# Autodesk Inventor assembly: ASY MSC 800 gills
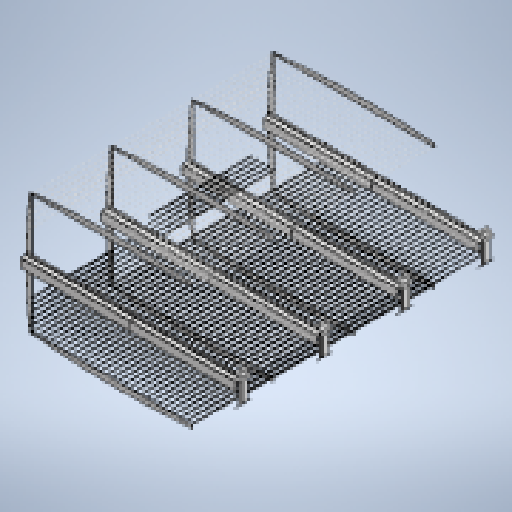
[picture p0: Inventor's stored thumbnail of the model, 512x512]
Saved by Autodesk Inventor 2025 (Build 290162010, 162A)
## iProperties
Created: 2024-08-31
Part Number: ASY MSC 800 gills
Document SubType Name: Assembly
Designer: pokla
Stock Number: ASY МОО 800 Жабры
Mass: 469810 g
Surface Area: 1.86943e+06 cm^2
Volume: 67870.7 cm^3
Density: 6.92212 g/cm^3
Author: pokla
## Documents named in this file (14)
- C:\Users\admin\YandexDisk-badmisterfox\домашниий пк\Inventor\Manturovo\Manturovo_Se-clar\ASY MSC 800 gills.iam
- C:\Users\admin\YandexDisk-badmisterfox\домашниий пк\Inventor\Manturovo\Manturovo_Se-clar\MSC 804 sheet gills.ipt
- C:\Users\admin\YandexDisk-badmisterfox\домашниий пк\Inventor\Manturovo\Manturovo_Se-clar\MSC 810 pillar gills.ipt
- C:\Users\admin\YandexDisk-badmisterfox\домашниий пк\Inventor\Manturovo\Manturovo_Se-clar\MSC 805 sheet gills.ipt
- C:\Users\admin\YandexDisk-badmisterfox\домашниий пк\Inventor\Manturovo\Manturovo_Se-clar\MSC 806 sheet gills.ipt
- C:\Users\admin\YandexDisk-badmisterfox\домашниий пк\Inventor\Manturovo\Manturovo_Se-clar\MSC 807 sheet gills.ipt
- C:\Users\admin\YandexDisk-badmisterfox\домашниий пк\Inventor\Manturovo\Manturovo_Se-clar\MSC 808 sheet gills.ipt
- C:\Users\admin\YandexDisk-badmisterfox\домашниий пк\Inventor\Manturovo\Manturovo_Se-clar\MSC 809 sheet gills.ipt
- C:\Users\admin\YandexDisk-badmisterfox\домашниий пк\Inventor\Manturovo\Manturovo_Se-clar\MSC 813 wall support gills.ipt
- C:\Users\admin\YandexDisk-badmisterfox\домашниий пк\Inventor\Manturovo\Manturovo_Se-clar\MSC 811 pillar gills.ipt
- C:\Users\admin\YandexDisk-badmisterfox\домашниий пк\Inventor\Manturovo\Manturovo_Se-clar\MSC 814 string for sheets gills.ipt
- C:\Users\admin\YandexDisk-badmisterfox\домашниий пк\Inventor\Manturovo\Manturovo_Se-clar\MSC 812 top support gills.ipt
- C:\Users\admin\YandexDisk-badmisterfox\домашниий пк\Inventor\Manturovo\Manturovo_Se-clar\MSC 803 sheet gills.ipt
- C:\Users\admin\YandexDisk-badmisterfox\домашниий пк\Inventor\Manturovo\Manturovo_Se-clar\ASY MSC 800.1 gills base.iam
## Components (272 placed, 13 different names)
1. MSC 0203 sheet gills:1 — Angle:2, Tangent:8, Tangent:9, Flush:15, Flush:19
2. MSC 0204 sheet gills:1 — Angle:3, Tangent:10, Tangent:11, Flush:15, Flush:16
3. MSC 0205 sheet gills:1 — Angle:4, Tangent:12, Tangent:13, Flush:16, Flush:17
4. MSC 0206 sheet gills:1 — Angle:5, Tangent:17, Tangent:18, Flush:17, Flush:18
5. MSC 0207 sheet gills:1 — Angle:6, Tangent:19, Tangent:20, Flush:18
6. MSC 814 string for sheets gills:143 — Rigid:40
7. MSC 814 string for sheets gills:152 — Rigid:24
8. MSC 814 string for sheets gills:371
9. MSC 814 string for sheets gills:372
10. MSC 814 string for sheets gills:373
11. MSC 814 string for sheets gills:374
12. MSC 814 string for sheets gills:375
13. MSC 814 string for sheets gills:2 — Rigid:12
14. MSC 0201 sheet gills:1 — Rigid:33, Angle:2, Angle:3, Angle:4, Angle:5, Angle:6, Tangent:14, Tangent:15, Tangent:16, Flush:19, Flush:24
15. MSC 804 sheet gills:1 — Rigid:33
16. MSC 814 string for sheets gills:1 — Rotational:1
17. MSC 814 string for sheets gills:3 — Rotational:2, Tangent:23
18. MSC 814 string for sheets gills:376 — Rotational:3, Tangent:21, Tangent:22
19. MSC 0201 sheet gills:30 — Tangent:21, Tangent:23, Flush:24
20. MSC 804 sheet gills:30 — Tangent:22
21. MSC 814 string for sheets gills:377
22. MSC 0201 sheet gills:2
23. MSC 804 sheet gills:2
24. MSC 814 string for sheets gills:378
25. MSC 814 string for sheets gills:379
26. MSC 814 string for sheets gills:380
27. MSC 0201 sheet gills:31
28. MSC 804 sheet gills:31
29. MSC 814 string for sheets gills:381
30. MSC 0201 sheet gills:3
31. MSC 804 sheet gills:3
32. MSC 814 string for sheets gills:382
33. MSC 814 string for sheets gills:383
34. MSC 814 string for sheets gills:384
35. MSC 0201 sheet gills:32
36. MSC 804 sheet gills:32
37. MSC 814 string for sheets gills:385
38. MSC 0201 sheet gills:4
39. MSC 804 sheet gills:4
40. MSC 814 string for sheets gills:386
41. MSC 814 string for sheets gills:387
42. MSC 814 string for sheets gills:388
43. MSC 0201 sheet gills:33
44. MSC 804 sheet gills:33
45. MSC 814 string for sheets gills:389
46. MSC 0201 sheet gills:5
47. MSC 804 sheet gills:5
48. MSC 814 string for sheets gills:390
49. MSC 814 string for sheets gills:391
50. MSC 814 string for sheets gills:392
51. MSC 0201 sheet gills:34
52. MSC 804 sheet gills:34
53. MSC 814 string for sheets gills:393
54. MSC 0201 sheet gills:6
55. MSC 804 sheet gills:6
56. MSC 814 string for sheets gills:394
57. MSC 814 string for sheets gills:395
58. MSC 814 string for sheets gills:396
59. MSC 0201 sheet gills:35
60. MSC 804 sheet gills:35
61. MSC 814 string for sheets gills:397
62. MSC 0201 sheet gills:7
63. MSC 804 sheet gills:7
64. MSC 814 string for sheets gills:398
65. MSC 814 string for sheets gills:399
66. MSC 814 string for sheets gills:400
67. MSC 0201 sheet gills:36
68. MSC 804 sheet gills:36
69. MSC 814 string for sheets gills:401
70. MSC 0201 sheet gills:8
71. MSC 804 sheet gills:8
72. MSC 814 string for sheets gills:402
73. MSC 814 string for sheets gills:403
74. MSC 814 string for sheets gills:404
75. MSC 0201 sheet gills:37
76. MSC 804 sheet gills:37
77. MSC 814 string for sheets gills:405
78. MSC 0201 sheet gills:9
79. MSC 804 sheet gills:9
80. MSC 814 string for sheets gills:406
81. MSC 814 string for sheets gills:407
82. MSC 814 string for sheets gills:408
83. MSC 0201 sheet gills:38
84. MSC 804 sheet gills:38
85. MSC 814 string for sheets gills:409
86. MSC 0201 sheet gills:10
87. MSC 804 sheet gills:10
88. MSC 814 string for sheets gills:410
89. MSC 814 string for sheets gills:411
90. MSC 814 string for sheets gills:412
91. MSC 0201 sheet gills:39
92. MSC 804 sheet gills:39
93. MSC 814 string for sheets gills:413
94. MSC 0201 sheet gills:11
95. MSC 804 sheet gills:11
96. MSC 814 string for sheets gills:414
97. MSC 814 string for sheets gills:415
98. MSC 814 string for sheets gills:416
99. MSC 0201 sheet gills:40
100. MSC 804 sheet gills:40
101. MSC 814 string for sheets gills:417
102. MSC 0201 sheet gills:12
103. MSC 804 sheet gills:12
104. MSC 814 string for sheets gills:418
105. MSC 814 string for sheets gills:419
106. MSC 814 string for sheets gills:420
107. MSC 0201 sheet gills:41
108. MSC 804 sheet gills:41
109. MSC 814 string for sheets gills:421
110. MSC 0201 sheet gills:13
111. MSC 804 sheet gills:13
112. MSC 814 string for sheets gills:422
113. MSC 814 string for sheets gills:423
114. MSC 814 string for sheets gills:424
115. MSC 0201 sheet gills:42
116. MSC 804 sheet gills:42
117. MSC 814 string for sheets gills:425
118. MSC 0201 sheet gills:14
119. MSC 804 sheet gills:14
120. MSC 814 string for sheets gills:426
121. MSC 814 string for sheets gills:427
122. MSC 814 string for sheets gills:428
123. MSC 0201 sheet gills:43
124. MSC 804 sheet gills:43
125. MSC 814 string for sheets gills:429
126. MSC 0201 sheet gills:15
127. MSC 804 sheet gills:15
128. MSC 814 string for sheets gills:430
129. MSC 814 string for sheets gills:431
130. MSC 814 string for sheets gills:432
131. MSC 0201 sheet gills:44
132. MSC 804 sheet gills:44
133. MSC 814 string for sheets gills:433
134. MSC 0201 sheet gills:16
135. MSC 804 sheet gills:16
136. MSC 814 string for sheets gills:434
137. MSC 814 string for sheets gills:435
138. MSC 814 string for sheets gills:436
139. MSC 0201 sheet gills:45
140. MSC 804 sheet gills:45
141. MSC 814 string for sheets gills:437
142. MSC 0201 sheet gills:17
143. MSC 804 sheet gills:17
144. MSC 814 string for sheets gills:438
145. MSC 814 string for sheets gills:439
146. MSC 814 string for sheets gills:440
147. MSC 0201 sheet gills:46
148. MSC 804 sheet gills:46
149. MSC 814 string for sheets gills:441
150. MSC 0201 sheet gills:18
151. MSC 804 sheet gills:18
152. MSC 814 string for sheets gills:442
153. MSC 814 string for sheets gills:443
154. MSC 814 string for sheets gills:444
155. MSC 0201 sheet gills:47
156. MSC 804 sheet gills:47
157. MSC 814 string for sheets gills:445
158. MSC 0201 sheet gills:19
159. MSC 804 sheet gills:19
160. MSC 814 string for sheets gills:446
161. MSC 814 string for sheets gills:447
162. MSC 814 string for sheets gills:448
163. MSC 0201 sheet gills:48
164. MSC 804 sheet gills:48
165. MSC 814 string for sheets gills:449
166. MSC 0201 sheet gills:20
167. MSC 804 sheet gills:20
168. MSC 814 string for sheets gills:450
169. MSC 814 string for sheets gills:451
170. MSC 814 string for sheets gills:452
171. MSC 0201 sheet gills:49
172. MSC 804 sheet gills:49
173. MSC 814 string for sheets gills:453
174. MSC 0201 sheet gills:21
175. MSC 804 sheet gills:21
176. MSC 814 string for sheets gills:454
177. MSC 814 string for sheets gills:455
178. MSC 814 string for sheets gills:456
179. MSC 0201 sheet gills:50
180. MSC 804 sheet gills:50
181. MSC 814 string for sheets gills:457
182. MSC 0201 sheet gills:22
183. MSC 804 sheet gills:22
184. MSC 814 string for sheets gills:458
185. MSC 814 string for sheets gills:459
186. MSC 814 string for sheets gills:460
187. MSC 0201 sheet gills:51
188. MSC 804 sheet gills:51
189. MSC 814 string for sheets gills:461
190. MSC 0201 sheet gills:23
191. MSC 804 sheet gills:23
192. MSC 814 string for sheets gills:462
193. MSC 814 string for sheets gills:463
194. MSC 814 string for sheets gills:464
195. MSC 0201 sheet gills:52
196. MSC 804 sheet gills:52
197. MSC 814 string for sheets gills:465
198. MSC 0201 sheet gills:24
199. MSC 804 sheet gills:24
200. MSC 814 string for sheets gills:466
201. MSC 814 string for sheets gills:467
202. MSC 814 string for sheets gills:468
203. MSC 0201 sheet gills:53
204. MSC 804 sheet gills:53
205. MSC 814 string for sheets gills:469
206. MSC 0201 sheet gills:25
207. MSC 804 sheet gills:25
208. MSC 814 string for sheets gills:470
209. MSC 814 string for sheets gills:471
210. MSC 814 string for sheets gills:472
211. MSC 0201 sheet gills:54
212. MSC 804 sheet gills:54
213. MSC 814 string for sheets gills:473
214. MSC 0201 sheet gills:26
215. MSC 804 sheet gills:26
216. MSC 814 string for sheets gills:474
217. MSC 814 string for sheets gills:475
218. MSC 814 string for sheets gills:476
219. MSC 0201 sheet gills:55
220. MSC 804 sheet gills:55
221. MSC 814 string for sheets gills:477
222. MSC 0201 sheet gills:27
223. MSC 804 sheet gills:27
224. MSC 814 string for sheets gills:478
225. MSC 814 string for sheets gills:479
226. MSC 814 string for sheets gills:480
227. MSC 0201 sheet gills:56
228. MSC 804 sheet gills:56
229. MSC 814 string for sheets gills:481
230. MSC 0201 sheet gills:28
231. MSC 804 sheet gills:28
232. MSC 814 string for sheets gills:482
233. MSC 814 string for sheets gills:483
234. MSC 814 string for sheets gills:484
235. MSC 0201 sheet gills:57
236. MSC 804 sheet gills:57
237. MSC 814 string for sheets gills:485
238. MSC 0201 sheet gills:29
239. MSC 804 sheet gills:29
240. MSC 814 string for sheets gills:486
241. MSC 814 string for sheets gills:487
242. MSC 814 string for sheets gills:488
243. MSC 0201 sheet gills:58
244. MSC 804 sheet gills:58
245. MSC 813 wall support gills:1 — Rigid:12, Rigid:30, Tangent:14, Tangent:15
246. MSC 812 top support gills:1 — Rigid:28, Rigid:30, Tangent:8, Tangent:9, Tangent:10, Tangent:11, Tangent:12, Tangent:13, Tangent:17, Tangent:18, Tangent:19, Tangent:20, Rigid:40
247. MSC 811 pillar gills:1 — Rigid:28, Rigid:29
248. MSC 812 top support gills:2 — Rigid:24, Rigid:29, Rigid:31
249. MSC 813 wall support gills:2 — Rigid:31, Rotational:3
250. MSC 810 pillar gills:1 — Rotational:1, Rotational:2, Tangent:16
251. ASY MSC 800.1 gills base:1 [sub-assembly]
252. MSC 813 wall support gills:4
253. MSC 812 top support gills:3
254. MSC 811 pillar gills:2
255. MSC 812 top support gills:4
256. MSC 813 wall support gills:5
257. MSC 810 pillar gills:2
258. ASY MSC 800.1 gills base:2 [sub-assembly]
259. MSC 813 wall support gills:6
260. MSC 812 top support gills:5
261. MSC 811 pillar gills:3
262. MSC 812 top support gills:6
263. MSC 813 wall support gills:7
264. MSC 810 pillar gills:3
265. ASY MSC 800.1 gills base:3 [sub-assembly]
266. MSC 813 wall support gills:8
267. MSC 812 top support gills:7
268. MSC 811 pillar gills:4
269. MSC 812 top support gills:8
270. MSC 813 wall support gills:9
271. MSC 810 pillar gills:4
272. ASY MSC 800.1 gills base:4 [sub-assembly]
## Component patterns: (6 elements, first: MSC 814 string for sheets gills:152), (29 elements, first: MSC 814 string for sheets gills:2 + MSC 0201 sheet gills:1 + MSC 804 sheet gills:1 + MSC 814 string for sheets gills:1 + MSC 814 string for sheets gills:3 + MSC 814 string for sheets gills:376 + MSC 0201 sheet gills:30 + MSC 804 sheet gills:30), (4 elements, first: MSC 813 wall support gills:1 + MSC 812 top support gills:1 + MSC 811 pillar gills:1 + MSC 812 top support gills:2 + MSC 813 wall support gills:2 + MSC 810 pillar gills:1 + ASY MSC 800.1 gills base:1)
## Relationships (46: Tangent 16, WeldJoint 10, Flush 9, Angle 5, Mate 3, RevoluteJoint 3)
- [WeldJoint]: MSC 811 pillar gills:1 ↔ MSC 810 pillar gills:1
- [Flush]: MSC 810 pillar gills:1 ↔ ASY MSC 800.1 gills base:1
- [Mate]: MSC 810 pillar gills:1 ↔ ASY MSC 800.1 gills base:1
- [Flush] (5 mm): MSC 810 pillar gills:1 ↔ ASY MSC 800.1 gills base:1
- Rigid:12 [WeldJoint] (-5 mm): MSC 814 string for sheets gills:2 ↔ MSC 813 wall support gills:1
- [Mate]: ASY MSC 800.1 gills base:1
- [Mate]: ASY MSC 800.1 gills base:1
- [Flush]: ASY MSC 800.1 gills base:1
- Rigid:24 [WeldJoint] (-5 mm): MSC 814 string for sheets gills:152 ↔ MSC 812 top support gills:2
- Rigid:28 [WeldJoint]: MSC 812 top support gills:1 ↔ MSC 811 pillar gills:1
- Rigid:29 [WeldJoint]: MSC 811 pillar gills:1 ↔ MSC 812 top support gills:2
- Rigid:30 [WeldJoint]: MSC 813 wall support gills:1 ↔ MSC 812 top support gills:1
- Rigid:31 [WeldJoint]: MSC 812 top support gills:2 ↔ MSC 813 wall support gills:2
- Rotational:1 [RevoluteJoint] (5 mm): MSC 814 string for sheets gills:1 ↔ MSC 810 pillar gills:1
- Rotational:2 [RevoluteJoint] (-5 mm): MSC 814 string for sheets gills:3 ↔ MSC 810 pillar gills:1
- Rigid:33 [WeldJoint] (-10 mm): MSC 0201 sheet gills:1 ↔ MSC 804 sheet gills:1
- Angle:2 (0 deg): MSC 0203 sheet gills:1 ↔ MSC 0201 sheet gills:1
- Angle:3 (0 deg): MSC 0204 sheet gills:1 ↔ MSC 0201 sheet gills:1
- Angle:4 (0 deg): MSC 0205 sheet gills:1 ↔ MSC 0201 sheet gills:1
- Angle:5 (0 deg): MSC 0206 sheet gills:1 ↔ MSC 0201 sheet gills:1
- Angle:6 (0 deg): MSC 0207 sheet gills:1 ↔ MSC 0201 sheet gills:1
- Tangent:8: MSC 0203 sheet gills:1 ↔ MSC 812 top support gills:1
- Tangent:9: MSC 0203 sheet gills:1 ↔ MSC 812 top support gills:1
- Tangent:10: MSC 0204 sheet gills:1 ↔ MSC 812 top support gills:1
- Tangent:11: MSC 0204 sheet gills:1 ↔ MSC 812 top support gills:1
- Tangent:12: MSC 0205 sheet gills:1 ↔ MSC 812 top support gills:1
- Tangent:13: MSC 0205 sheet gills:1 ↔ MSC 812 top support gills:1
- Tangent:14: MSC 0201 sheet gills:1 ↔ MSC 813 wall support gills:1
- Tangent:15: MSC 0201 sheet gills:1 ↔ MSC 813 wall support gills:1
- Tangent:16: MSC 0201 sheet gills:1 ↔ MSC 810 pillar gills:1
- Tangent:17: MSC 0206 sheet gills:1 ↔ MSC 812 top support gills:1
- Tangent:18: MSC 0206 sheet gills:1 ↔ MSC 812 top support gills:1
- Tangent:19: MSC 0207 sheet gills:1 ↔ MSC 812 top support gills:1
- Tangent:20: MSC 0207 sheet gills:1 ↔ MSC 812 top support gills:1
- Flush:15: MSC 0203 sheet gills:1 ↔ MSC 0204 sheet gills:1
- Flush:16: MSC 0204 sheet gills:1 ↔ MSC 0205 sheet gills:1
- Flush:17: MSC 0205 sheet gills:1 ↔ MSC 0206 sheet gills:1
- Flush:18: MSC 0206 sheet gills:1 ↔ MSC 0207 sheet gills:1
- Flush:19: MSC 0203 sheet gills:1 ↔ MSC 0201 sheet gills:1
- Rigid:40 [WeldJoint] (5 mm): MSC 814 string for sheets gills:143 ↔ MSC 812 top support gills:1
- Rotational:3 [RevoluteJoint] (-5 mm): MSC 814 string for sheets gills:376 ↔ MSC 813 wall support gills:2
- [WeldJoint] (-10 mm): MSC 0201 sheet gills:30 ↔ MSC 804 sheet gills:30
- Tangent:21: MSC 814 string for sheets gills:376 ↔ MSC 0201 sheet gills:30
- Tangent:22: MSC 814 string for sheets gills:376 ↔ MSC 804 sheet gills:30
- Tangent:23: MSC 814 string for sheets gills:3 ↔ MSC 0201 sheet gills:30
- Flush:24: MSC 0201 sheet gills:1 ↔ MSC 0201 sheet gills:30
